# Autodesk Inventor assembly: componente1
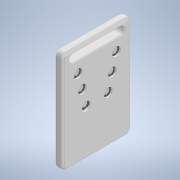
[picture p0: Inventor's stored thumbnail of the model, 180x180]
Saved by Autodesk Inventor 2021 (Build 250183000, 183)
## iProperties
Created: 2021-10-12
Part Number: componente1
Document SubType Name: Assembly
Designer: gonza
Author: gonza
## Documents named in this file (6)
- C:\Users\USUARIO\Dropbox\Mi PC (LAPTOP-MNA512CM)\Desktop\componente1.iam
- C:\Users\USUARIO\Dropbox\Mi PC (LAPTOP-MNA512CM)\Desktop\Biodiseño\MainShellCase.ipt
- C:\Users\USUARIO\Dropbox\Mi PC (LAPTOP-MNA512CM)\Desktop\Biodiseño\Woofer.iam
- C:\Users\USUARIO\Dropbox\Mi PC (LAPTOP-MNA512CM)\Desktop\Biodiseño\CorrectedFinal.ipt
- C:\Users\USUARIO\Dropbox\Mi PC (LAPTOP-MNA512CM)\Desktop\Biodiseño\reMinified.ipt
- C:\Users\USUARIO\Dropbox\Mi PC (LAPTOP-MNA512CM)\Desktop\Biodiseño\MainWorkingElectronic\AIP\Tubos y tuberías\MainWorkingElectronic.Conductos de tubos y tuberías.iam
## Components (12 placed, 5 different names)
1. Woofer:1 [sub-assembly] — Coincidencia:8, Coincidencia:9
2. MainShellCase:1 — Flush:1, Mate:1, Coincidencia:8, Coincidencia:9, Coincidencia:10, Coincidencia:11, Coincidencia:12, Coincidencia:13, Coincidencia:14, Coincidencia:15, Coincidencia:16, Coincidencia:17, Coincidencia:18, Coincidencia:19, Coincidencia:20, Coincidencia:21, Coincidencia:22, Coincidencia:23, Coincidencia:24, Coincidencia:25, Coincidencia:26, Coincidencia:27, Coincidencia:29, Coincidencia:30
3. Woofer:2 [sub-assembly] — Coincidencia:12, Coincidencia:15
4. Woofer:3 [sub-assembly] — Coincidencia:14, Coincidencia:18
5. Woofer:4 [sub-assembly] — Coincidencia:13, Coincidencia:17
6. Woofer:5 [sub-assembly] — Coincidencia:10, Coincidencia:16
7. Woofer:6 [sub-assembly] — Coincidencia:11, Coincidencia:19
8. CorrectedFinal:1 — Coincidencia:29, Coincidencia:30
9. reMinified:1 — Coincidencia:21, Coincidencia:27, Coincidencia:28
10. reMinified:2 — Coincidencia:22, Coincidencia:25, Coincidencia:26
11. reMinified:3 — Coincidencia:20, Coincidencia:23, Coincidencia:24, Coincidencia:28
12. Conductos de tubos y tuberías [sub-assembly]
## Relationships (25: Mate 24, Flush 1)
- Flush:1: MainShellCase:1
- Mate:1: MainShellCase:1
- Coincidencia:8 [Mate]: Woofer:1 ↔ MainShellCase:1
- Coincidencia:9 [Mate]: Woofer:1 ↔ MainShellCase:1
- Coincidencia:10 [Mate]: MainShellCase:1 ↔ Woofer:5
- Coincidencia:11 [Mate]: MainShellCase:1 ↔ Woofer:6
- Coincidencia:12 [Mate]: MainShellCase:1 ↔ Woofer:2
- Coincidencia:13 [Mate]: MainShellCase:1 ↔ Woofer:4
- Coincidencia:14 [Mate]: MainShellCase:1 ↔ Woofer:3
- Coincidencia:15 [Mate]: MainShellCase:1 ↔ Woofer:2
- Coincidencia:16 [Mate]: MainShellCase:1 ↔ Woofer:5
- Coincidencia:17 [Mate]: MainShellCase:1 ↔ Woofer:4
- Coincidencia:18 [Mate]: MainShellCase:1 ↔ Woofer:3
- Coincidencia:19 [Mate]: MainShellCase:1 ↔ Woofer:6
- Coincidencia:20 [Mate]: MainShellCase:1 ↔ reMinified:3
- Coincidencia:21 [Mate]: MainShellCase:1 ↔ reMinified:1
- Coincidencia:22 [Mate]: MainShellCase:1 ↔ reMinified:2
- Coincidencia:23 [Mate] (15 mm): MainShellCase:1 ↔ reMinified:3
- Coincidencia:24 [Mate] (10 mm): MainShellCase:1 ↔ reMinified:3
- Coincidencia:25 [Mate] (15 mm): MainShellCase:1 ↔ reMinified:2
- Coincidencia:26 [Mate] (10 mm): MainShellCase:1 ↔ reMinified:2
- Coincidencia:27 [Mate] (10 mm): MainShellCase:1 ↔ reMinified:1
- Coincidencia:28 [Mate] (17.125 mm): reMinified:1 ↔ reMinified:3
- Coincidencia:29 [Mate]: MainShellCase:1 ↔ CorrectedFinal:1
- Coincidencia:30 [Mate]: MainShellCase:1 ↔ CorrectedFinal:1
